# Autodesk Inventor assembly: case
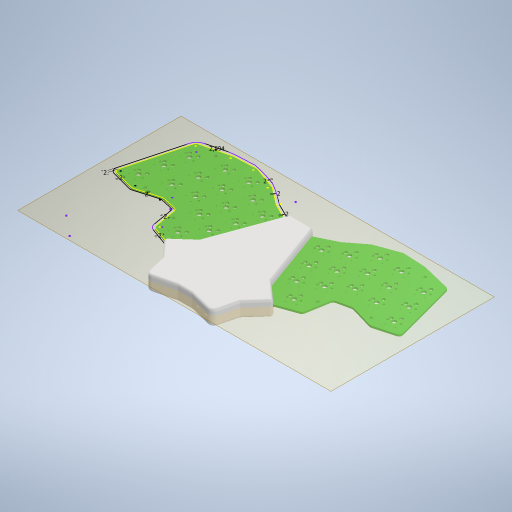
[picture p0: Inventor's stored thumbnail of the model, 512x512]
Saved by Autodesk Inventor 2024 (Build 280153000, 153)
## iProperties
Created: 2024-09-29
Part Number: case
Document SubType Name: Assembly
Designer: nikla
Author: nikla
## Documents named in this file (5)
- C:\Users\nikla\OneDrive\Keyboards\Blavinge\case\case.iam
- C:\Users\nikla\OneDrive\Keyboards\Blavinge\kicad\blavinge\blavinge.iam
- C:\Users\nikla\OneDrive\Keyboards\Blavinge\case\middle_top.ipt
- C:\Users\nikla\OneDrive\Keyboards\Blavinge\case\middle_bottom.ipt
- C:\Users\nikla\OneDrive\Keyboards\Blavinge\case\left_top.ipt
## Components (4 placed, 4 different names)
1. blavinge:1 [sub-assembly] — Fluchtend:1, Fluchtend:2, Fluchtend:3, Fluchtend:4
2. middle_top:1 — Fluchtend:1
3. middle_bottom:1 — Fluchtend:2
4. left_top:1 — Fluchtend:3, Fluchtend:4
## Relationships (4: Flush 4)
- Fluchtend:1 [Flush]: blavinge:1 ↔ middle_top:1
- Fluchtend:2 [Flush]: blavinge:1 ↔ middle_bottom:1
- Fluchtend:3 [Flush]: blavinge:1 ↔ left_top:1
- Fluchtend:4 [Flush]: blavinge:1 ↔ left_top:1
